# Autodesk Inventor assembly: Motor_ZSB
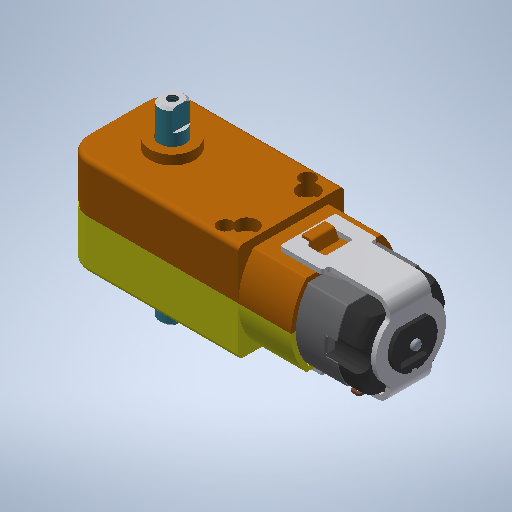
[picture p0: Inventor's stored thumbnail of the model, 512x512]
Saved by Autodesk Inventor 2025.1 (Build 291241000, 241)
## iProperties
Created: 2022-10-31
Part Number: Motor_ZSB
Material: Generisch
Document SubType Name: Assembly
Designer: RP
Author: RP
## Documents named in this file (11)
- C:\Users\Erik\Erik\Hochschule\3. Semester\CAD\CAD-Paspa\Useless Box\_Useless_Box\Motor_ZSB.iam
- C:\Users\Erik\Erik\Hochschule\3. Semester\CAD\CAD-Paspa\Useless Box\_Useless_Box\Motor_Unterseite.ipt
- C:\Users\Erik\Erik\Hochschule\3. Semester\CAD\CAD-Paspa\Useless Box\_Useless_Box\Motor.ipt
- C:\Users\Erik\Erik\Hochschule\3. Semester\CAD\CAD-Paspa\Useless Box\_Useless_Box\Motor_Achse.ipt
- C:\Users\Erik\Erik\Hochschule\3. Semester\CAD\CAD-Paspa\Useless Box\_Useless_Box\Motor_Ausgangswelle.ipt
- C:\Users\Erik\Erik\Hochschule\3. Semester\CAD\CAD-Paspa\Useless Box\_Useless_Box\Motor_Oberseite.ipt
- C:\Users\Erik\Erik\Hochschule\3. Semester\CAD\CAD-Paspa\Useless Box\_Useless_Box\Motor_Sicherungsblech.ipt
- C:\Users\Erik\Erik\Hochschule\3. Semester\CAD\CAD-Paspa\Useless Box\_Useless_Box\Motor_Stirnradpaar_2_3.ipt
- C:\Users\Erik\Erik\Hochschule\3. Semester\CAD\CAD-Paspa\Useless Box\_Useless_Box\Motor_Stirnradpaar_3_4.ipt
- C:\Users\Erik\Erik\Hochschule\3. Semester\CAD\CAD-Paspa\Useless Box\_Useless_Box\Motor_Tellerrad.ipt
- C:\Users\Erik\Erik\Hochschule\3. Semester\CAD\CAD-Paspa\Useless Box\_Useless_Box\Motor_Schraube.ipt
## Components (11 placed, 10 different names)
1. Motor_Unterseite:1 — Mate:1, Flush:1, Mate:2, Insert:1, Insert:2, Insert:3, Insert:5, Angle:1, Mate:4, Angle:2, Insert:10, Insert:11
2. Motor_Ausgangswelle:1 — Insert:1, Insert:4, Mate:3, Angle:5
3. Motor_Achse:1 — Insert:2
4. Motor_Stirnradpaar_3_4:1 — Insert:3, Insert:6
5. Motor_Stirnradpaar_2_3:1 — Insert:4
6. Motor:1 — Insert:5, Angle:1, Insert:7, Angle:3, Angle:5
7. Motor_Tellerrad:1 — Insert:6
8. Motor_Oberseite:1 — Mate:3, Mate:4, Angle:2
9. Motor_Schraube:1 — Insert:10, Angle:4
10. Motor_Schraube:2 — Insert:11
11. Motor_Sicherungsblech:1 — Insert:7, Angle:3, Angle:4
## Relationships (19: Insert 9, Angle 5, Mate 4, Flush 1)
- Mate:1: Motor_Unterseite:1
- Flush:1: Motor_Unterseite:1
- Mate:2: Motor_Unterseite:1
- Insert:1: Motor_Unterseite:1 ↔ Motor_Ausgangswelle:1
- Insert:2: Motor_Unterseite:1 ↔ Motor_Achse:1
- Insert:3: Motor_Unterseite:1 ↔ Motor_Stirnradpaar_3_4:1
- Insert:4: Motor_Ausgangswelle:1 ↔ Motor_Stirnradpaar_2_3:1
- Insert:5: Motor_Unterseite:1 ↔ Motor:1
- Angle:1 (0 deg): Motor_Unterseite:1 ↔ Motor:1
- Insert:6 (0.3 mm): Motor_Stirnradpaar_3_4:1 ↔ Motor_Tellerrad:1
- Mate:3: Motor_Ausgangswelle:1 ↔ Motor_Oberseite:1
- Mate:4: Motor_Unterseite:1 ↔ Motor_Oberseite:1
- Angle:2 (0 deg): Motor_Unterseite:1 ↔ Motor_Oberseite:1
- Insert:7: Motor:1 ↔ Motor_Sicherungsblech:1
- Angle:3 (180 deg): Motor:1 ↔ Motor_Sicherungsblech:1
- Insert:10: Motor_Unterseite:1 ↔ Motor_Schraube:1
- Angle:4 (0 deg): Motor_Schraube:1 ↔ Motor_Sicherungsblech:1
- Insert:11: Motor_Unterseite:1 ↔ Motor_Schraube:2
- Angle:5 (0 deg): Motor_Ausgangswelle:1 ↔ Motor:1
